# Autodesk Inventor assembly: Rover
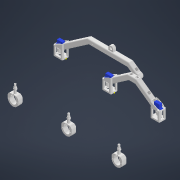
[picture p0: Inventor's stored thumbnail of the model, 180x180]
Saved by Autodesk Inventor 2021 (Build 250183000, 183)
## iProperties
Created: 2021-01-03
Part Number: Rover
Document SubType Name: Assembly
Designer: laure
Author: laure
## Documents named in this file (10)
- E:\Projects\Rover\Rover.iam
- E:\Projects\Rover\Rocker_hinten.ipt
- E:\Projects\Rover\Rocker_vorne.ipt
- E:\Projects\Rover\Servohalterung.ipt
- E:\Projects\Rover\Bogie.ipt
- E:\Projects\Rover\MicroServo.ipt
- E:\Projects\Rover\Übersetzungsbox.ipt
- E:\Projects\Rover\Zahnrad_innen.ipt
- E:\Projects\Rover\Motorhalterung.ipt
- E:\Projects\Rover\Zahnrad_außen.ipt
## Components (21 placed, 9 different names)
1. Fahrwerk_rocker_hinten:1 — Passend:3, Passend:4, Drehbar:1
2. Fahrwerk_rocker_vorne:1 — Passend:1, Passend:2, Passend:3, Passend:4
3. Servohalterung:1 — Passend:1, Passend:2, Passend:9, Passend:10, Passend:15
4. Servohalterung:2 — Passend:5, Passend:6, Passend:11, Passend:12, Passend:16
5. Servohalterung:3 — Passend:7, Passend:8, Passend:13, Passend:14, Passend:17
6. Fahrwerk_bogie:1 — Passend:5, Passend:6, Passend:7, Passend:8, Drehbar:1
7. MicroServo:1 — Passend:9, Passend:10, Drehbar:4
8. MicroServo:2 — Passend:11, Passend:12, Drehbar:3
9. MicroServo:3 — Passend:13, Passend:14, Drehbar:2
10. Übersetzungsbox:1 — Passend:15
11. Übersetzungsbox:2 — Passend:16
12. Übersetzungsbox:3 — Passend:17
13. Zahnrad_innen:1 — Drehbar:4, Passend:18
14. Zahnrad_innen:2 — Drehbar:3, Passend:19
15. Zahnrad_innen:3 — Drehbar:2, Passend:20
16. Fahrwerk_motorhalterung:1
17. Fahrwerk_motorhalterung:2
18. Fahrwerk_motorhalterung:3
19. Zahnrad_außen:1 — Passend:18
20. Zahnrad_außen:2 — Passend:19
21. Zahnrad_außen:3 — Passend:20
## Relationships (24: Mate 20, RevoluteJoint 4)
- Passend:1 [Mate]: Fahrwerk_rocker_vorne:1 ↔ Servohalterung:1
- Passend:2 [Mate]: Fahrwerk_rocker_vorne:1 ↔ Servohalterung:1
- Passend:3 [Mate]: Fahrwerk_rocker_hinten:1 ↔ Fahrwerk_rocker_vorne:1
- Passend:4 [Mate]: Fahrwerk_rocker_hinten:1 ↔ Fahrwerk_rocker_vorne:1
- Passend:5 [Mate]: Servohalterung:2 ↔ Fahrwerk_bogie:1
- Passend:6 [Mate]: Servohalterung:2 ↔ Fahrwerk_bogie:1
- Passend:7 [Mate]: Servohalterung:3 ↔ Fahrwerk_bogie:1
- Passend:8 [Mate]: Servohalterung:3 ↔ Fahrwerk_bogie:1
- Drehbar:1 [RevoluteJoint]: Fahrwerk_rocker_hinten:1 ↔ Fahrwerk_bogie:1
- Passend:9 [Mate]: Servohalterung:1 ↔ MicroServo:1
- Passend:10 [Mate]: Servohalterung:1 ↔ MicroServo:1
- Passend:11 [Mate]: Servohalterung:2 ↔ MicroServo:2
- Passend:12 [Mate]: Servohalterung:2 ↔ MicroServo:2
- Passend:13 [Mate]: Servohalterung:3 ↔ MicroServo:3
- Passend:14 [Mate]: Servohalterung:3 ↔ MicroServo:3
- Passend:15 [Mate]: Servohalterung:1 ↔ Übersetzungsbox:1
- Passend:16 [Mate]: Servohalterung:2 ↔ Übersetzungsbox:2
- Passend:17 [Mate]: Servohalterung:3 ↔ Übersetzungsbox:3
- Drehbar:2 [RevoluteJoint]: MicroServo:3 ↔ Zahnrad_innen:3
- Drehbar:3 [RevoluteJoint]: MicroServo:2 ↔ Zahnrad_innen:2
- Drehbar:4 [RevoluteJoint]: MicroServo:1 ↔ Zahnrad_innen:1
- Passend:18 [Mate]: Zahnrad_innen:1 ↔ Zahnrad_außen:1
- Passend:19 [Mate]: Zahnrad_innen:2 ↔ Zahnrad_außen:2
- Passend:20 [Mate]: Zahnrad_innen:3 ↔ Zahnrad_außen:3
